# Autodesk Inventor assembly: koilicek
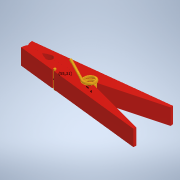
[picture p0: Inventor's stored thumbnail of the model, 180x180]
Saved by Autodesk Inventor 2022 (Build 260153000, 153)
## iProperties
Created: 2021-05-30
Part Number: koilicek
Document SubType Name: Assembly
Designer: HP
Author: HP
## Documents named in this file (3)
- C:\Users\HP\OneDrive\Dokumenty\Inventor\modely\koilicek.iam
- C:\Users\HP\OneDrive\Dokumenty\Inventor\modely\kolik_drivko.ipt
- C:\Users\HP\OneDrive\Dokumenty\Inventor\modely\pruzina.ipt
## Components (3 placed, 2 different names)
1. kolik_drivko:1 — Proti sobě:1, Proti sobě:2, Proti sobě:3
2. kolik_drivko:2 — Stejný směr:1, Proti sobě:2
3. pruzina:1 — Stejný směr:2
## Relationships (5: Mate 3, Flush 2)
- Proti sobě:1 [Mate]: kolik_drivko:1
- Stejný směr:1 [Flush]: kolik_drivko:2
- Proti sobě:2 [Mate]: kolik_drivko:1 ↔ kolik_drivko:2
- Proti sobě:3 [Mate]: kolik_drivko:1
- Stejný směr:2 [Flush]: pruzina:1
